# Autodesk Inventor assembly: rear_bumper_mirrored
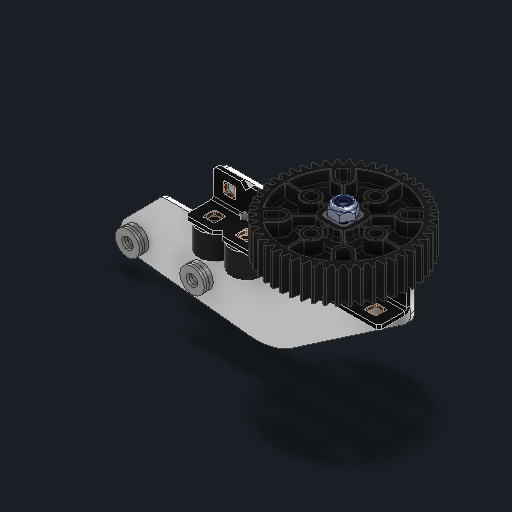
[picture p0: Inventor's stored thumbnail of the model, 512x512]
Saved by Autodesk Inventor 2024 (Build 280153000, 153)
## iProperties
Created: 2024-02-11
Part Number: rear_bumper_mirrored
Document SubType Name: Assembly
Designer: Averey Ku
Author: Averey Ku
## Documents named in this file (14)
- D:\vex_robotics\hardware\cad\vroomba_v0.1\chassis\drivebay\mirrored_parts\rear_bumper_mirrored.iam
- D:\vex_robotics\hardware\cad\vroomba_v0.1\chassis\drivebay\mirrored_parts\sled_mirrored.ipt
- D:\vex_robotics\hardware\cad\vroomba_v0.1\chassis\drivebay\mirrored_parts\Alu Angle 1x1x6_mirrored.ipt
- D:\vex_robotics\hardware\cad\VEX-CAD-Inventor-1.41\Motion\Spacers\Spacer Nylon .500 OD\NSpacer Black .500 OD x .375.ipt
- D:\vex_robotics\hardware\cad\VEX-CAD-Inventor-1.41\Motion\Spacers\Spacer Nylon .500 OD.ipt
- D:\vex_robotics\hardware\cad\VEX-CAD-Inventor-1.41\Motion\Spacers\Washer Steel\SWasher .375 OD x .062500.ipt
- D:\vex_robotics\hardware\cad\VEX-CAD-Inventor-1.41\Motion\Spacers\Washer Steel.ipt
- D:\vex_robotics\hardware\cad\VEX-CAD-Inventor-1.41\Motion\Spacers\Washer Teflon\TWasher .375 OD x .04000.ipt
- D:\vex_robotics\hardware\cad\VEX-CAD-Inventor-1.41\Motion\Spacers\Washer Teflon.ipt
- D:\vex_robotics\hardware\cad\vroomba_v0.1\chassis\drivebay\mirrored_parts\Nut Keps_mirrored.ipt
- D:\vex_robotics\hardware\cad\VEX-CAD-Inventor-1.41\Motion\Spacers\Spacer Nylon .375 OD\NSpacer .375 OD x .375.ipt
- D:\vex_robotics\hardware\cad\VEX-CAD-Inventor-1.41\Motion\Spacers\Spacer Nylon .375 OD.ipt
- D:\vex_robotics\hardware\cad\vroomba_v0.1\chassis\drivebay\mirrored_parts\HS 48T Gear, No Insert_mirrored.iam
- D:\vex_robotics\hardware\cad\vroomba_v0.1\chassis\drivebay\mirrored_parts\Nut Thin Nylock_mirrored.ipt
## Components (14 placed, 9 different names)
1. sled_mirrored:1 — Mate:1, Insert:1, Insert:9, Insert:8
2. Alu Angle 1x1x6_mirrored:1 — Mate:1, Insert:1, Insert:2, Insert:3, Insert:13
3. NSpacer Black .500 OD x .375:1 — Insert:2
4. NSpacer Black .500 OD x .375:2 — Insert:3
5. SWasher .375 OD x .062500:1 — Insert:9, Insert:5
6. TWasher .375 OD x .04000:1 — Insert:4
7. TWasher .375 OD x .04000:2 — Insert:5, Insert:4
8. SWasher .375 OD x .062500:2 — Insert:8, Insert:7
9. TWasher .375 OD x .04000:3 — Insert:6
10. TWasher .375 OD x .04000:4 — Insert:7, Insert:6
11. Nut Keps_mirrored:1 — Insert:13, Insert:10
12. NSpacer .375 OD x .375:1 — Insert:10, Insert:11
13. HS 48T Gear, No Insert_mirrored:1 [sub-assembly] — Insert:11, Insert:12
14. Nut Thin Nylock_mirrored:1 — Insert:12
## Relationships (14: Insert 13, Mate 1)
- Mate:1: sled_mirrored:1 ↔ Alu Angle 1x1x6_mirrored:1
- Insert:1: sled_mirrored:1 ↔ Alu Angle 1x1x6_mirrored:1
- Insert:2: Alu Angle 1x1x6_mirrored:1 ↔ NSpacer Black .500 OD x .375:1
- Insert:3: Alu Angle 1x1x6_mirrored:1 ↔ NSpacer Black .500 OD x .375:2
- Insert:9: sled_mirrored:1 ↔ SWasher .375 OD x .062500:1
- Insert:5: SWasher .375 OD x .062500:1 ↔ TWasher .375 OD x .04000:2
- Insert:4: TWasher .375 OD x .04000:1 ↔ TWasher .375 OD x .04000:2
- Insert:8: sled_mirrored:1 ↔ SWasher .375 OD x .062500:2
- Insert:7: SWasher .375 OD x .062500:2 ↔ TWasher .375 OD x .04000:4
- Insert:6: TWasher .375 OD x .04000:3 ↔ TWasher .375 OD x .04000:4
- Insert:13: Alu Angle 1x1x6_mirrored:1 ↔ Nut Keps_mirrored:1
- Insert:10: Nut Keps_mirrored:1 ↔ NSpacer .375 OD x .375:1
- Insert:11: NSpacer .375 OD x .375:1 ↔ HS 48T Gear, No Insert_mirrored:1
- Insert:12: HS 48T Gear, No Insert_mirrored:1 ↔ Nut Thin Nylock_mirrored:1
